# Autodesk Inventor assembly: head
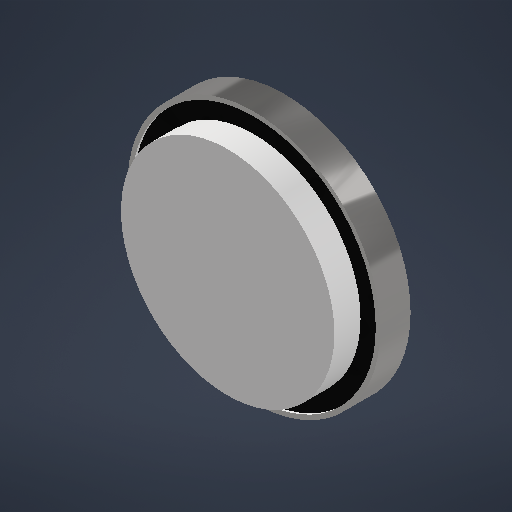
[picture p0: Inventor's stored thumbnail of the model, 512x512]
Saved by Autodesk Inventor 2026.1 (Build 301233000, 233)
## iProperties
Created: 2026-04-17
Part Number: head
Document SubType Name: Assembly
Designer: aaron
Author: aaron
## Documents named in this file (3)
- D:\work\loopandpixel\openworkoutsystem\cad\v5\head.iam
- D:\work\loopandpixel\openworkoutsystem\cad\v5\bearings\bearing_58x45x7.ipt
- D:\work\loopandpixel\openworkoutsystem\cad\v5\head_innter_top.ipt
## Components (2 placed, 2 different names)
1. bearing_58x45x7:1 — Insert:1
2. head_innter_top:1 — Insert:1
## Relationships (1: Insert 1)
- Insert:1: bearing_58x45x7:1 ↔ head_innter_top:1
